# Autodesk Inventor assembly: Assembly1
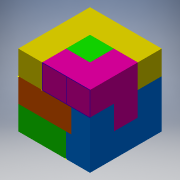
[picture p0: Inventor's stored thumbnail of the model, 180x180]
Saved by Autodesk Inventor 2016 (Build 200138000, 138)
## iProperties
Created: 2017-10-02
Part Number: Assembly1
Document SubType Name: Assembly
Designer: sun01147
Author: sun01147
## Documents named in this file (6)
- E:\IED7_SunT\IED7_Practice\IED7_Puzzle Cube\Assembly1.iam
- E:\IED7_SunT\IED7_Practice\IED7_Puzzle Cube\IED7_Sun_PuzzleCubeBlue.ipt
- E:\IED7_SunT\IED7_Practice\IED7_Puzzle Cube\IED7_Sun_PuzzleCubeOrange.ipt
- E:\IED7_SunT\IED7_Practice\IED7_Puzzle Cube\IED7_Sun_PuzzleCubePink.ipt
- E:\IED7_SunT\IED7_Practice\IED7_Puzzle Cube\IED7_Sun_PuzzleCubeYellow.ipt
- E:\IED7_SunT\IED7_Practice\IED7_Puzzle Cube\IED7_Sun_PuzzleCubeGreen_new.ipt
## Components (5 placed, 5 different names)
1. IED7_Sun_PuzzleCubeBlue:1 — Mate:2, Mate:3, Mate:4, Mate:6, Mate:7, Flush:1
2. IED7_Sun_PuzzleCubePink:1 — Mate:2, Mate:3, Mate:4, Mate:5, Flush:2
3. IED7_Sun_PuzzleCubeYellow:1 — Mate:5, Mate:6, Flush:3
4. IED7_Sun_PuzzleCubeOrange:3 — Mate:8, Mate:9, Flush:3, Flush:4
5. IED7_Sun_PuzzleCubeGreen_new:1 — Mate:7, Flush:1, Flush:2, Mate:8, Mate:9, Flush:4
## Relationships (12: Mate 8, Flush 4)
- Mate:2: IED7_Sun_PuzzleCubeBlue:1 ↔ IED7_Sun_PuzzleCubePink:1
- Mate:3: IED7_Sun_PuzzleCubeBlue:1 ↔ IED7_Sun_PuzzleCubePink:1
- Mate:4: IED7_Sun_PuzzleCubeBlue:1 ↔ IED7_Sun_PuzzleCubePink:1
- Mate:5: IED7_Sun_PuzzleCubePink:1 ↔ IED7_Sun_PuzzleCubeYellow:1
- Mate:6: IED7_Sun_PuzzleCubeBlue:1 ↔ IED7_Sun_PuzzleCubeYellow:1
- Mate:7: IED7_Sun_PuzzleCubeBlue:1 ↔ IED7_Sun_PuzzleCubeGreen_new:1
- Flush:1: IED7_Sun_PuzzleCubeBlue:1 ↔ IED7_Sun_PuzzleCubeGreen_new:1
- Flush:2: IED7_Sun_PuzzleCubePink:1 ↔ IED7_Sun_PuzzleCubeGreen_new:1
- Mate:8: IED7_Sun_PuzzleCubeOrange:3 ↔ IED7_Sun_PuzzleCubeGreen_new:1
- Mate:9: IED7_Sun_PuzzleCubeOrange:3 ↔ IED7_Sun_PuzzleCubeGreen_new:1
- Flush:3: IED7_Sun_PuzzleCubeYellow:1 ↔ IED7_Sun_PuzzleCubeOrange:3
- Flush:4: IED7_Sun_PuzzleCubeOrange:3 ↔ IED7_Sun_PuzzleCubeGreen_new:1
